# Autodesk Inventor assembly: Suporte de Talheres
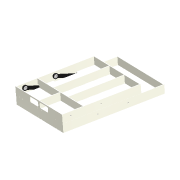
[picture p0: Inventor's stored thumbnail of the model, 180x180]
Saved by Autodesk Inventor 2020 (Build 240168000, 168)
## iProperties
Created: 2021-09-22
Part Number: Suporte de Talheres
Document SubType Name: Assembly
Designer: pablo
Author: pablo
## Documents named in this file (5)
- C:\Google Drive\Pablo Arquivos\Projetos\Utilidades Domesticas\Talheres\Suporte de Talheres.iam
- C:\Google Drive\Pablo Arquivos\Projetos\Utilidades Domesticas\Talheres\Suporte Superior.iam
- C:\Google Drive\Pablo Arquivos\Projetos\Utilidades Domesticas\Talheres\Cursor.ipt
- C:\Google Drive\Pablo Arquivos\Projetos\Utilidades Domesticas\Talheres\Suporte Inferior.iam
- C:\Google Drive\Pablo Arquivos\Projetos\Utilidades Domesticas\Talheres\Third\AIS2019\SKF_619_6-2Z.iam
## Components (14 placed, 4 different names)
1. Suporte Superior:1 [sub-assembly] — Mate:13, Mate:14, Mate:23, Mate:24, Mate:25
2. Cursor:1 — Mate:1, Mate:2, Mate:4
3. Cursor:2 — Mate:9, Mate:10, Mate:11
4. Cursor:3 — Mate:15, Mate:16, Mate:21
5. Cursor:4 — Mate:17, Mate:18, Mate:22, Mate:25
6. Suporte Inferior:1 [sub-assembly] — Mate:3, Mate:4, Mate:8, Mate:9, Mate:12, Mate:19, Mate:20, Mate:21, Mate:22
7. SKF_619_6-2Z:1 [sub-assembly] — Mate:18, Mate:24
8. SKF_619_6-2Z:2 [sub-assembly] — Mate:17, Mate:20
9. SKF_619_6-2Z:3 [sub-assembly] — Mate:15, Mate:23
10. SKF_619_6-2Z:4 [sub-assembly] — Mate:8, Mate:10, Mate:12
11. SKF_619_6-2Z:5 [sub-assembly] — Mate:2, Mate:14
12. SKF_619_6-2Z:6 [sub-assembly] — Mate:16, Mate:19
13. SKF_619_6-2Z:7 [sub-assembly] — Mate:1, Mate:3
14. SKF_619_6-2Z:8 [sub-assembly] — Mate:11, Mate:13
## Relationships (22: Mate 22)
- Mate:1: Cursor:1 ↔ SKF_619_6-2Z:7
- Mate:2: Cursor:1 ↔ SKF_619_6-2Z:5
- Mate:3: Suporte Inferior:1 ↔ SKF_619_6-2Z:7
- Mate:4: Cursor:1 ↔ Suporte Inferior:1
- Mate:8: Suporte Inferior:1 ↔ SKF_619_6-2Z:4
- Mate:9: Cursor:2 ↔ Suporte Inferior:1
- Mate:10: Cursor:2 ↔ SKF_619_6-2Z:4
- Mate:11: Cursor:2 ↔ SKF_619_6-2Z:8
- Mate:12: Suporte Inferior:1 ↔ SKF_619_6-2Z:4
- Mate:13: Suporte Superior:1 ↔ SKF_619_6-2Z:8
- Mate:14: Suporte Superior:1 ↔ SKF_619_6-2Z:5
- Mate:15: Cursor:3 ↔ SKF_619_6-2Z:3
- Mate:16: Cursor:3 ↔ SKF_619_6-2Z:6
- Mate:17: Cursor:4 ↔ SKF_619_6-2Z:2
- Mate:18: Cursor:4 ↔ SKF_619_6-2Z:1
- Mate:19: Suporte Inferior:1 ↔ SKF_619_6-2Z:6
- Mate:20: Suporte Inferior:1 ↔ SKF_619_6-2Z:2
- Mate:21: Cursor:3 ↔ Suporte Inferior:1
- Mate:22: Cursor:4 ↔ Suporte Inferior:1
- Mate:23: Suporte Superior:1 ↔ SKF_619_6-2Z:3
- Mate:24: Suporte Superior:1 ↔ SKF_619_6-2Z:1
- Mate:25: Suporte Superior:1 ↔ Cursor:4
